# Autodesk Inventor assembly: ballShooterV02
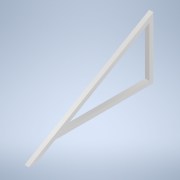
[picture p0: Inventor's stored thumbnail of the model, 180x180]
Saved by Autodesk Inventor 2020.2 (Build 242310000, 310)
## iProperties
Created: 2020-01-16
Part Number: ballShooterV02
Document SubType Name: Assembly
Designer: robst
Author: robst
## Documents named in this file (4)
- C:\git\CAD-Development\robSteele\2020LongRobotBase\ballShooterV02.iam
- C:\git\CAD-Development\robSteele\2020BallTriggerMechanism\aluminumBallHandlerBase.ipt
- C:\git\CAD-Development\robSteele\2020BallTriggerMechanism\aluminumBallHandlerBackLeg.ipt
- C:\git\CAD-Development\robSteele\2020BallTriggerMechanism\aluminumBallHandlerHypotenuse.ipt
## Components (3 placed, 3 different names)
1. aluminumBallHandlerBase:1 — Mate:1, Mate:2, Flush:1
2. aluminumBallHandlerBackLeg:1 — Mate:1, Mate:2, Flush:1, Mate:3, Mate:4, Flush:2
3. aluminumBallHandlerHypotenuse:1 — Mate:3, Mate:4, Flush:2
## Relationships (6: Mate 4, Flush 2)
- Mate:1: aluminumBallHandlerBase:1 ↔ aluminumBallHandlerBackLeg:1
- Mate:2: aluminumBallHandlerBase:1 ↔ aluminumBallHandlerBackLeg:1
- Flush:1: aluminumBallHandlerBase:1 ↔ aluminumBallHandlerBackLeg:1
- Mate:3: aluminumBallHandlerBackLeg:1 ↔ aluminumBallHandlerHypotenuse:1
- Mate:4: aluminumBallHandlerBackLeg:1 ↔ aluminumBallHandlerHypotenuse:1
- Flush:2: aluminumBallHandlerBackLeg:1 ↔ aluminumBallHandlerHypotenuse:1
